# Autodesk Inventor assembly: Main
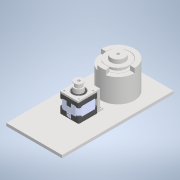
[picture p0: Inventor's stored thumbnail of the model, 180x180]
Saved by Autodesk Inventor 2022.3 (Build 263350000, 350)
## iProperties
Created: 2022-05-27
Part Number: Main
Document SubType Name: Assembly
Designer: Mlees
Author: Mlees
## Documents named in this file (7)
- D:\504Engineering\Project_0000\Main.iam
- D:\504Engineering\Project_0000\Designs\Design_5\Downloaded_Parts\127076899-9-stp-mtrl-14034_nema_14\stp-mtrl-14034.ipt
- D:\504Engineering\Project_0000\Designs\Design_5\Created_Parts\GT2 20T.ipt
- D:\504Engineering\Project_0000\Designs\Design_5\Created_Parts\Base.ipt
- D:\504Engineering\Project_0000\Designs\Design_5\Created_Parts\Motor_Mount.ipt
- D:\504Engineering\Project_0000\Designs\Design_5\Created_Parts\GT2 60T.ipt
- D:\504Engineering\Project_0000\Designs\Design_5\Downloaded_Parts\4668K334_Permanently Lubricated Stainless Steel Ball Bearing 688-2RS.ipt
## Components (7 placed, 6 different names)
1. stp-mtrl-14034:1 — Mate:1, Mate:2, Mate:6, Mate:7
2. GT2 20T:1 — Mate:1, Mate:2
3. Base:1 — Mate:5, Mate:8, Mate:9, Mate:12, Mate:13, Mate:14, Mate:15, Mate:16, Mate:17
4. Motor_Mount:1 — Mate:5, Mate:6, Mate:7, Mate:16, Mate:17
5. GT2 60T:1 — Mate:8, Mate:9
6. 4668K334_Permanently Lubricated Stainless Steel Ball Bearing 688-2RS:1 — Mate:12, Mate:13
7. 4668K334_Permanently Lubricated Stainless Steel Ball Bearing 688-2RS:2 — Mate:14, Mate:15
## Relationships (13: Mate 13)
- Mate:1: stp-mtrl-14034:1 ↔ GT2 20T:1
- Mate:2 (1 mm): stp-mtrl-14034:1 ↔ GT2 20T:1
- Mate:5: Base:1 ↔ Motor_Mount:1
- Mate:6: stp-mtrl-14034:1 ↔ Motor_Mount:1
- Mate:7: stp-mtrl-14034:1 ↔ Motor_Mount:1
- Mate:8: Base:1 ↔ GT2 60T:1
- Mate:9: Base:1 ↔ GT2 60T:1
- Mate:12: Base:1 ↔ 4668K334_Permanently Lubricated Stainless Steel Ball Bearing 688-2RS:1
- Mate:13: Base:1 ↔ 4668K334_Permanently Lubricated Stainless Steel Ball Bearing 688-2RS:1
- Mate:14: Base:1 ↔ 4668K334_Permanently Lubricated Stainless Steel Ball Bearing 688-2RS:2
- Mate:15: Base:1 ↔ 4668K334_Permanently Lubricated Stainless Steel Ball Bearing 688-2RS:2
- Mate:16: Base:1 ↔ Motor_Mount:1
- Mate:17: Base:1 ↔ Motor_Mount:1
